# Autodesk Inventor assembly: Assembly1
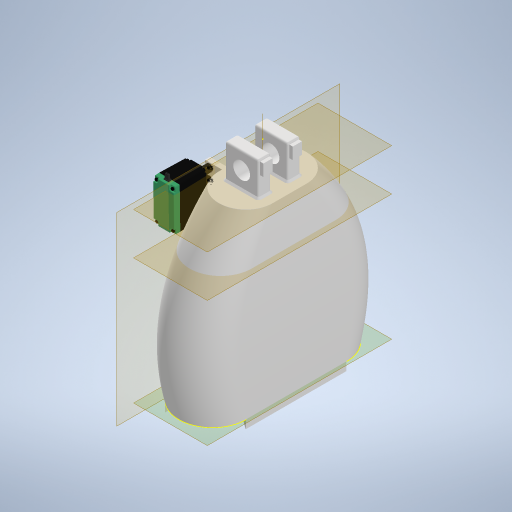
[picture p0: Inventor's stored thumbnail of the model, 512x512]
Saved by Autodesk Inventor 2023 (Build 270158000, 158)
## iProperties
Created: 2024-12-06
Part Number: Assembly1
Document SubType Name: Assembly
Designer: 1ZHUSAM
Author: 1ZHUSAM
## Documents named in this file (3)
- G:\tekdezrob\VEX Parts Library 2016-20241107T143136Z-001\Assembly1.iam
- G:\tekdezrob\VEX Parts Library 2016-20241107T143136Z-001\Part13.ipt
- G:\tekdezrob\VEX Parts Library 2016-20241107T143136Z-001\VEX Parts Library 2016\Imperial\Motion\393 Motor.iam
## Components (2 placed, 2 different names)
1. Part13:1 — Mate:1
2. 393 Motor:1 [sub-assembly] — Mate:1
## Relationships (1: Mate 1)
- Mate:1: Part13:1 ↔ 393 Motor:1
